# Autodesk Inventor assembly: 21-09x-PHANTOM-HRDSET
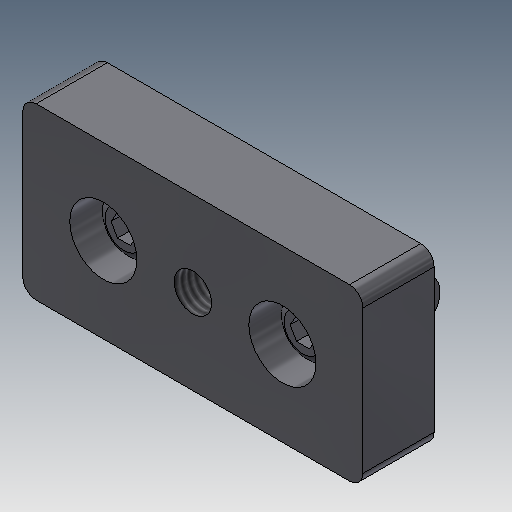
[picture p0: Inventor's stored thumbnail of the model, 512x512]
Saved by Autodesk Inventor 2018.3 (Build 223284000, 284)
## iProperties
Created: 2004-11-19
Part Number: 21-09x-PHANTOM-HRDSET
Document SubType Name: Assembly
Designer: Autodesk, Inc.
Manufacturer: Standard
Standards Organization: Custom
Description: PHANTOM, CASTER MOUNT, HARDWARE SET
Catalog Web Link: http://www.parker.com/ead/cm1.asp?cmid=809
Vendor: PARKER IPS
Mass: 363.586 g
Surface Area: 145.109 cm^2
Volume: 46.3757 cm^3
Density: 7.84 g/cm^3
CAGE: 1LJX3
Dept. ID: Product Design
Description #2: ---
Finish #1: ---
Finish #2: ---
Material ID: ---
Project Number: ---
Author: Autodesk, Inc.
## Documents named in this file (7)
- C:\AVAInvAPI\Workspace\Test Station\Components\21-09x_Caster_Mnt_Phantom.iam
- C:\AVAInvAPI\Workspace\Test Station\Components\24-118-8.ipt
- C:\AVAInvAPI\Workspace\Test Station\Components\21-002.ipt
- C:\AVAInvAPI\Workspace\Test Station\Components\20-058.ipt
- C:\Users\kelleyb.ADS\Desktop\Samples MIGRATED 2009 224 RTM_1\Standard Parts\Test Station Content\Fastners\2X-YYY-ZZ IPS Screws.ipt
- C:\Users\kelleyb.ADS\Desktop\Samples MIGRATED 2009 224 RTM_1\Standard Parts\Test Station Content\Corners, Gussets, and Mounting Plates\21-XXX Mounting Plates.ipt
- C:\Users\kelleyb.ADS\Desktop\Samples MIGRATED 2009 224 RTM_1\Standard Parts\Test Station Content\Fastners\20-XXX TSlot Nuts.ipt
## Components (5 placed, 3 different names)
1. 24-118-8:1
2. 24-118-8:2
3. 21-002:1
4. 20-058:1
5. 20-058:2
## Relationships (8: Mate 4, Insert 2, Angle 2)
- [Insert]: 24-118-8:1 ↔ 21-002:1
- [Mate]: 24-118-8:1 ↔ 20-058:1
- [Insert]: 24-118-8:2 ↔ 21-002:1
- [Mate]: 24-118-8:2 ↔ 20-058:2
- [Mate] (4.5 mm): 21-002:1 ↔ 20-058:2
- [Mate] (4.5 mm): 21-002:1 ↔ 20-058:1
- [Angle] (0 deg): 21-002:1 ↔ 20-058:2
- [Angle] (0 deg): 21-002:1 ↔ 20-058:1
